# Autodesk Inventor assembly: Assembly_Cube_Mirror_v2
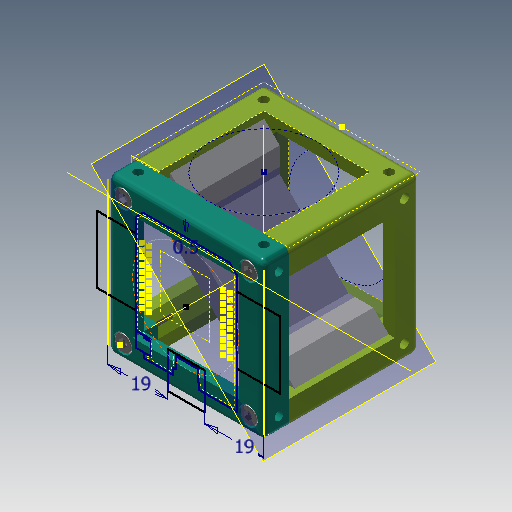
[picture p0: Inventor's stored thumbnail of the model, 512x512]
Saved by Autodesk Inventor 2019 (Build 230136000, 136)
## iProperties
Created: 2019-07-22
Part Number: Assembly_Cube_Mirror_v2
Document SubType Name: Assembly
Designer: diederichbenedict
Author: diederichbenedict
## Documents named in this file (3)
- C:\Users\diederichbenedict\Dropbox\Dokumente\Promotion\PROJECTS\UC2\02_CAD\INVENTOR\uc2_v2\Assembly_Cube_Mirror_v2.iam
- C:\Users\diederichbenedict\Dropbox\Dokumente\Promotion\PROJECTS\UC2\02_CAD\INVENTOR\uc2_v2\Assembly_Cube_empty_1x1_v2.iam
- C:\Users\diederichbenedict\Dropbox\Dokumente\Promotion\PROJECTS\UC2\02_CAD\INVENTOR\uc2_v2\20_Cube_Insert_Mirror_Holder_v2.ipt
## Components (2 placed, 2 different names)
1. Assembly_Cube_empty_1x1_v2:1 [sub-assembly] — Flush:1, Mate:1, Mate:2
2. 20_Cube_Insert_Mirror_Holder_v2:1 — Flush:1, Mate:1, Mate:2
## Relationships (3: Mate 2, Flush 1)
- Flush:1: Assembly_Cube_empty_1x1_v2:1 ↔ 20_Cube_Insert_Mirror_Holder_v2:1
- Mate:1: Assembly_Cube_empty_1x1_v2:1 ↔ 20_Cube_Insert_Mirror_Holder_v2:1
- Mate:2: Assembly_Cube_empty_1x1_v2:1 ↔ 20_Cube_Insert_Mirror_Holder_v2:1
